# Autodesk Inventor assembly: CAN
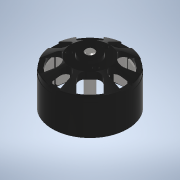
[picture p0: Inventor's stored thumbnail of the model, 180x180]
Saved by Autodesk Inventor 2022 (Build 260153000, 153)
## iProperties
Created: 2022-07-25
Part Number: CAN
Document SubType Name: Assembly
Designer: Nathan Cai
Author: Nathan Cai
## Documents named in this file (5)
- C:\Users\Nathan Cai\Documents\Inventor\Asorted Parts\Aerosky MC4230 630KV\CAN.iam
- C:\Users\Nathan Cai\Documents\Inventor\Asorted Parts\Aerosky MC4230 630KV\CAN - LOWER.ipt
- C:\Users\Nathan Cai\Documents\Inventor\Asorted Parts\Aerosky MC4230 630KV\MAGNETS.ipt
- C:\Users\Nathan Cai\Documents\Inventor\Asorted Parts\Aerosky MC4230 630KV\TOP.ipt
- C:\Users\Nathan Cai\Documents\Inventor\Asorted Parts\Aerosky MC4230 630KV\SHAFT.ipt
## Components (17 placed, 4 different names)
1. CAN - LOWER:1 — Tangent:1, Tangent:2, Flush:1, Mate:1, Mate:2
2. TOP:1 — Mate:1, Mate:2, Mate:3, Mate:4
3. SHAFT:1 — Mate:3, Mate:4
4. MAGNETS:1 — Tangent:1, Tangent:2, Flush:1
5. MAGNETS:2
6. MAGNETS:3
7. MAGNETS:4
8. MAGNETS:5
9. MAGNETS:6
10. MAGNETS:7
11. MAGNETS:8
12. MAGNETS:9
13. MAGNETS:10
14. MAGNETS:11
15. MAGNETS:12
16. MAGNETS:13
17. MAGNETS:14
## Component patterns: (14 elements, first: MAGNETS:1)
## Relationships (7: Mate 4, Tangent 2, Flush 1)
- Tangent:1: CAN - LOWER:1 ↔ MAGNETS:1
- Tangent:2: CAN - LOWER:1 ↔ MAGNETS:1
- Flush:1 (0.5 mm): CAN - LOWER:1 ↔ MAGNETS:1
- Mate:1: CAN - LOWER:1 ↔ TOP:1
- Mate:2: CAN - LOWER:1 ↔ TOP:1
- Mate:3: TOP:1 ↔ SHAFT:1
- Mate:4: TOP:1 ↔ SHAFT:1
